# Autodesk Inventor assembly: Сборка2
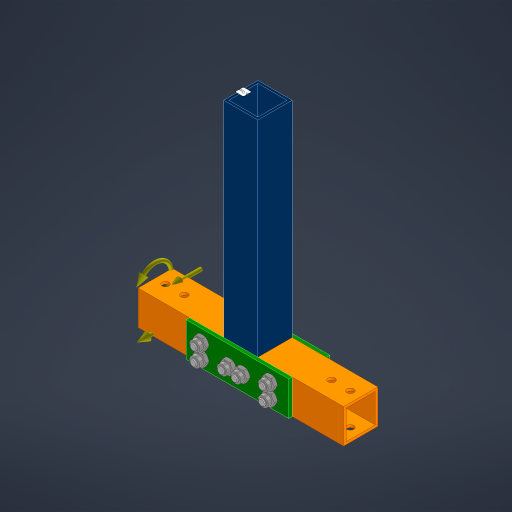
[picture p0: Inventor's stored thumbnail of the model, 512x512]
Saved by Autodesk Inventor 2024 (Build 280153000, 153)
## iProperties
Created: 2023-04-17
Part Number: Сборка2
Document SubType Name: Assembly
Designer: user
Mass: 85.5465 g
Surface Area: 459.769 cm^2
Volume: 34.3914 cm^3
Density: 2.48744 g/cm^3
Author: user
## Documents named in this file (12)
- D:\Docs\Robot\3d\tests\var2\Сборка2.iam
- D:\Docs\Robot\3d\tests\var2\1.ipt
- D:\Docs\Robot\3d\base\plate.ipt
- D:\Docs\Robot\3d\base\side_section.ipt
- C:\Users\user\Documents\Inventor\Content Center Files\R2024\ru-RU\DIN 7985 (H)\DIN 7985 (H) - M4x30-H.ipt
- C:\Users\user\Documents\Inventor\Content Center Files\R2024\ru-RU\DIN 985\DIN 985 - M4.ipt
- D:\Docs\Robot\3d\tests\var2\Сборка2\AIP\FEA\eb2vbnxfk.fins
- D:\Docs\Robot\3d\tests\var2\Сборка2\AIP\FEA\eb2vbnxfk.fsat
- D:\Docs\Robot\3d\tests\var2\Сборка2\AIP\FEA\eb2vbnxfk.ftes
- D:\Docs\Robot\3d\tests\var2\Сборка2\AIP\FEA\eb2vbnxfk.fwiz
- D:\Docs\Robot\3d\tests\var2\Сборка2\AIP\FEA\eb2vbnxj4.fmsh
- D:\Docs\Robot\3d\tests\var2\Сборка2\AIP\FEA\eb2vbnxj5.fres
## Components (17 placed, 5 different names)
1. 1:1 — Вставка:1, Вставка:2, Вставка:3, Вставка:4
2. plate:1 — Вставка:1, Вставка:2, Вставка:5, Вставка:6, Вставка:7, Вставка:8, Вставка:9, Вставка:10, Вставка:11, Вставка:12, Вставка:13, Вставка:14
3. plate:2 — Вставка:3, Вставка:4, Вставка:15, Вставка:16, Вставка:17, Вставка:18, Вставка:19, Вставка:20
4. side_section:1 — Вставка:5, Вставка:6
5. side_section:2 — Вставка:7, Вставка:8
6. DIN 7985 (H) M4x30-H:1 — Вставка:9
7. DIN 7985 (H) M4x30-H:2 — Вставка:10
8. DIN 7985 (H) M4x30-H:3 — Вставка:11
9. DIN 7985 (H) M4x30-H:4 — Вставка:12
10. DIN 7985 (H) M4x30-H:5 — Вставка:13
11. DIN 7985 (H) M4x30-H:6 — Вставка:14
12. DIN 985 - заменено на DIN EN ISO 10511 M4:1 — Вставка:19
13. DIN 985 - заменено на DIN EN ISO 10511 M4:2 — Вставка:17
14. DIN 985 - заменено на DIN EN ISO 10511 M4:3 — Вставка:15
15. DIN 985 - заменено на DIN EN ISO 10511 M4:4 — Вставка:20
16. DIN 985 - заменено на DIN EN ISO 10511 M4:5 — Вставка:18
17. DIN 985 - заменено на DIN EN ISO 10511 M4:6 — Вставка:16
## Relationships (20: Insert 20)
- Вставка:1 [Insert]: 1:1 ↔ plate:1
- Вставка:2 [Insert]: 1:1 ↔ plate:1
- Вставка:3 [Insert]: 1:1 ↔ plate:2
- Вставка:4 [Insert]: 1:1 ↔ plate:2
- Вставка:5 [Insert]: plate:1 ↔ side_section:1
- Вставка:6 [Insert]: plate:1 ↔ side_section:1
- Вставка:7 [Insert]: plate:1 ↔ side_section:2
- Вставка:8 [Insert]: plate:1 ↔ side_section:2
- Вставка:9 [Insert]: plate:1 ↔ DIN 7985 (H) M4x30-H:1
- Вставка:10 [Insert]: plate:1 ↔ DIN 7985 (H) M4x30-H:2
- Вставка:11 [Insert]: plate:1 ↔ DIN 7985 (H) M4x30-H:3
- Вставка:12 [Insert]: plate:1 ↔ DIN 7985 (H) M4x30-H:4
- Вставка:13 [Insert]: plate:1 ↔ DIN 7985 (H) M4x30-H:5
- Вставка:14 [Insert]: plate:1 ↔ DIN 7985 (H) M4x30-H:6
- Вставка:15 [Insert]: plate:2 ↔ DIN 985 - заменено на DIN EN ISO 10511 M4:3
- Вставка:16 [Insert]: plate:2 ↔ DIN 985 - заменено на DIN EN ISO 10511 M4:6
- Вставка:17 [Insert]: plate:2 ↔ DIN 985 - заменено на DIN EN ISO 10511 M4:2
- Вставка:18 [Insert]: plate:2 ↔ DIN 985 - заменено на DIN EN ISO 10511 M4:5
- Вставка:19 [Insert]: plate:2 ↔ DIN 985 - заменено на DIN EN ISO 10511 M4:1
- Вставка:20 [Insert]: plate:2 ↔ DIN 985 - заменено на DIN EN ISO 10511 M4:4
## Named parameters: sa_0 = 5000, sa_1 = 50000, sa_2 = 50000
note: some values were not read from the file. Shown as the stored number, unit unknown: "sa_0", "sa_1", "sa_2".
